# Autodesk Inventor assembly: Fuselage Structure Assembly
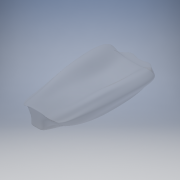
[picture p0: Inventor's stored thumbnail of the model, 180x180]
Saved by Autodesk Inventor 2018 (Build 220112000, 112)
## iProperties
Created: 2018-08-08
Part Number: Fuselage Structure Assembly
Document SubType Name: Assembly
Designer: Michael Gunderman
Author: Michael Gunderman
## Documents named in this file (2)
- C:\Users\Michael Gunderman\Documents\Special Projects\Echo 1\8-7-18\Echo-1-master\Echo 1\CAD work\Structures\Fuselage\Fuselage Structure Assembly.iam
- C:\Users\Michael Gunderman\Documents\Special Projects\Echo 1\8-7-18\Echo-1-master\Echo 1\CAD work\Preliminary Shapes\Generic Fuselage.ipt
## Components (1 placed, 1 different names)
1. Generic Fuselage:1 — Mate:1
## Relationships (1: Mate 1)
- Mate:1: Generic Fuselage:1
